# Autodesk Inventor assembly: SORTING Assembly
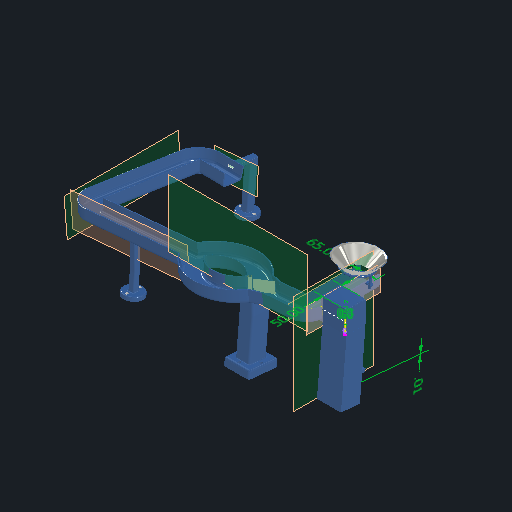
[picture p0: Inventor's stored thumbnail of the model, 512x512]
Saved by Autodesk Inventor 2026.2 (Build 302298010, 298A)
## iProperties
Created: 2026-04-17
Part Number: SORTING Assembly
Document SubType Name: Assembly
Designer: lenovo
Author: lenovo
## Documents named in this file (10)
- F:\Semester 4\Basics of Mechatronics\Final\SORTING Assembly.iam
- F:\Semester 4\Basics of Mechatronics\Final\path.ipt
- F:\Semester 4\Basics of Mechatronics\Final\Basket Holder 2 .ipt
- F:\Semester 4\Basics of Mechatronics\Final\Gate.ipt
- F:\Semester 4\Basics of Mechatronics\Final\IR_LM393_pin.ipt
- F:\Semester 4\Basics of Mechatronics\Final\basket.ipt
- F:\Semester 4\Basics of Mechatronics\Final\Cover of Sensors.ipt
- F:\Semester 4\Basics of Mechatronics\Final\00_마이크로 서보_SG90.ipt
- F:\Semester 4\Basics of Mechatronics\Final\Path (from sorting to storage).ipt
- F:\Semester 4\Basics of Mechatronics\Final\Base of Sorting.ipt
## Components (9 placed, 9 different names)
1. Path:1 — Mate:15, Mate:21, Mate:22, Mate:23, Mate:25, Mate:26, Mate:27, Mate:28, Mate:30, Mate:31, Mate:32
2. IR_LM393_pin:2 — Mate:15
3. Gate:2 — Mate:29, Mate:33, Mate:34, Mate:35, Mate:36
4. basket:4 — Mate:24
5. Basket Holder:1 — Mate:21, Mate:22, Mate:23, Mate:24, Mate:25
6. Cover of Sensors:2 — Mate:26, Mate:27, Mate:28
7. 00_마이크로 서보_SG90:1 — Mate:29, Mate:35, Mate:36
8. Path (from sorting to storage):1
9. Base of Sorting:1 — Mate:30, Mate:31, Mate:32, Mate:33, Mate:34
## Relationships (17: Mate 17)
- Mate:15 (2.3 mm): Path:1 ↔ IR_LM393_pin:2
- Mate:21: Path:1 ↔ Basket Holder:1
- Mate:22: Path:1 ↔ Basket Holder:1
- Mate:23: Path:1 ↔ Basket Holder:1
- Mate:24: basket:4 ↔ Basket Holder:1
- Mate:25: Path:1 ↔ Basket Holder:1
- Mate:26: Path:1 ↔ Cover of Sensors:2
- Mate:27: Path:1 ↔ Cover of Sensors:2
- Mate:28: Path:1 ↔ Cover of Sensors:2
- Mate:29: Gate:2 ↔ 00_마이크로 서보_SG90:1
- Mate:30: Path:1 ↔ Base of Sorting:1
- Mate:31: Path:1 ↔ Base of Sorting:1
- Mate:32: Path:1 ↔ Base of Sorting:1
- Mate:33: Gate:2 ↔ Base of Sorting:1
- Mate:34: Gate:2 ↔ Base of Sorting:1
- Mate:35: Gate:2 ↔ 00_마이크로 서보_SG90:1
- Mate:36: Gate:2 ↔ 00_마이크로 서보_SG90:1
## Named parameters: Finish1_Area = 3848.39, Finish1_Thickness = 0.05 mm, Finish2_Area = 991.841, Finish2_Thickness = 0.05 mm, Finish3_Area = 250.53, Finish3_Thickness = 0.05 mm, Finish4_Area = 21.7649, Finish4_Thickness = 0.05 mm, Finish5_Area = 0.424115, Finish5_Thickness = 0.05 mm, Finish6_Area = 1.92426, Finish6_Thickness = 0.05 mm
note: some values were not read from the file. Shown as the stored number, unit unknown: "Finish1_Area", "Finish2_Area", "Finish3_Area", "Finish4_Area", "Finish5_Area", "Finish6_Area".
